# Autodesk Inventor assembly: Giant-Snes-Gamepad
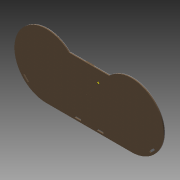
[picture p0: Inventor's stored thumbnail of the model, 180x180]
Saved by Autodesk Inventor 2014 SP1 (Build 180222100, 222)
## iProperties
Created: 2014-01-12
Part Number: Giant-Snes-Gamepad
Document SubType Name: Assembly
Designer: tuleu
Author: tuleu
## Documents named in this file (9)
- C:\Users\tuleu\Documents\giant-snes-gamepad\cad\Giant_Snes_Gamepad.iam
- C:\Users\tuleu\Documents\giant-snes-gamepad\cad\Base.ipt
- C:\Users\tuleu\Documents\giant-snes-gamepad\cad\Link.ipt
- C:\Users\tuleu\Documents\giant-snes-gamepad\cad\Square_Cell.iam
- C:\Users\tuleu\Documents\giant-snes-gamepad\cad\Trigger_Cell.iam
- C:\Users\tuleu\Documents\giant-snes-gamepad\cad\Foam_Left.ipt
- C:\Users\tuleu\Documents\giant-snes-gamepad\cad\Start_Cell.iam
- C:\Users\tuleu\Documents\giant-snes-gamepad\cad\Circle_Cell.iam
- C:\Users\tuleu\Documents\giant-snes-gamepad\cad\Foam_Right.ipt
## Components (19 placed, 8 different names)
1. Base:1 — Mate:1, Mate:2, Flush:1, Mate:3, Mate:5, Mate:6, Flush:3, Mate:15, Mate:16, Mate:17, Mate:18, Mate:20, Mate:21, Mate:22, Mate:24, Flush:22, Mate:29, Mate:31, Mate:32, Mate:33, Mate:35, Angle:1, Mate:37, Angle:2
2. Base:2 — Mate:1, Mate:2, Flush:1, Mate:3, Mate:4, Flush:2, Mate:10, Mate:11, Mate:12, Mate:13, Mate:27, Mate:28, Mate:30, Mate:34, Mate:38, Mate:39, Mate:40, Mate:41, Mate:42, Mate:43, Mate:46, Mate:47, Mate:48, Mate:49, Mate:50, Mate:51, Mate:53, Mate:54, Mate:55
3. Link:1 — Mate:4, Flush:2, Mate:12
4. Link:2 — Mate:5, Mate:10, Mate:14
5. Link:3 — Mate:6, Flush:3, Mate:11
6. Square_Cell:1 [sub-assembly] — Mate:17, Mate:19, Symmetry:2, Mate:20, Mate:23
7. Square_Cell:2 [sub-assembly] — Mate:15, Flush:21, Symmetry:1
8. Square_Cell:3 [sub-assembly] — Mate:16, Mate:19, Symmetry:2
9. Square_Cell:4 [sub-assembly] — Mate:18, Flush:21, Symmetry:1, Mate:21, Mate:22
10. Trigger_Cell:1 [sub-assembly] — Mate:24, Flush:22, Mate:29
11. Trigger_Cell:2 [sub-assembly] — Mate:27, Mate:28, Mate:30
12. Foam_Left:1 — Mate:31, Mate:32
13. Start_Cell:1 [sub-assembly] — Mate:33, Mate:36, Mate:37
14. Start_Cell:2 [sub-assembly] — Mate:34, Flush:23, Mate:39
15. Circle_Cell:1 [sub-assembly] — Mate:40, Mate:44, Mate:46, Mate:48
16. Circle_Cell:2 [sub-assembly] — Mate:41, Mate:45, Mate:47, Mate:50
17. Circle_Cell:3 [sub-assembly] — Mate:42, Mate:44, Mate:49
18. Circle_Cell:4 [sub-assembly] — Mate:43, Mate:45, Mate:51
19. Foam_Right:1 — Mate:53, Mate:54, Mate:55
## Relationships (59: Mate 49, Flush 6, Symmetry 2, Angle 2)
- Mate:1: Base:1 ↔ Base:2
- Mate:2: Base:1 ↔ Base:2
- Flush:1: Base:1 ↔ Base:2
- Mate:3: Base:1 ↔ Base:2
- Mate:4: Base:2 ↔ Link:1
- Mate:5: Base:1 ↔ Link:2
- Mate:6: Base:1 ↔ Link:3
- Flush:2: Base:2 ↔ Link:1
- Flush:3: Base:1 ↔ Link:3
- Mate:10: Base:2 ↔ Link:2
- Mate:11: Base:2 ↔ Link:3
- Mate:12: Base:2 ↔ Link:1
- Mate:13: Base:2
- Mate:14: Link:2
- Mate:15: Base:1 ↔ Square_Cell:2
- Mate:16: Base:1 ↔ Square_Cell:3
- Mate:17: Base:1 ↔ Square_Cell:1
- Mate:18: Base:1 ↔ Square_Cell:4
- Mate:19: Square_Cell:1 ↔ Square_Cell:3
- Flush:21: Square_Cell:2 ↔ Square_Cell:4
- Symmetry:1: Square_Cell:2 ↔ Square_Cell:4
- Symmetry:2: Square_Cell:1 ↔ Square_Cell:3
- Mate:20: Base:1 ↔ Square_Cell:1
- Mate:21: Base:1 ↔ Square_Cell:4
- Mate:22 (205 mm): Base:1 ↔ Square_Cell:4
- Mate:23 (-205 mm): Square_Cell:1
- Mate:24: Base:1 ↔ Trigger_Cell:1
- Mate:27: Base:2 ↔ Trigger_Cell:2
- Flush:22: Base:1 ↔ Trigger_Cell:1
- Mate:28: Base:2 ↔ Trigger_Cell:2
- Mate:29 (-400 mm): Base:1 ↔ Trigger_Cell:1
- Mate:30 (-400 mm): Base:2 ↔ Trigger_Cell:2
- Mate:31: Base:1 ↔ Foam_Left:1
- Mate:32: Base:1 ↔ Foam_Left:1
- Mate:33: Base:1 ↔ Start_Cell:1
- Mate:34: Base:2 ↔ Start_Cell:2
- Mate:35: Base:1
- Angle:1 (0 deg): Base:1
- Mate:36: Start_Cell:1
- Mate:37: Base:1 ↔ Start_Cell:1
- Mate:38: Base:2
- Angle:2 (0 deg): Base:1
- Flush:23: Start_Cell:2
- Mate:39: Base:2 ↔ Start_Cell:2
- Mate:40: Base:2 ↔ Circle_Cell:1
- Mate:41: Base:2 ↔ Circle_Cell:2
- Mate:42: Base:2 ↔ Circle_Cell:3
- Mate:43: Base:2 ↔ Circle_Cell:4
- Mate:44: Circle_Cell:1 ↔ Circle_Cell:3
- Mate:45: Circle_Cell:2 ↔ Circle_Cell:4
- Mate:46: Base:2 ↔ Circle_Cell:1
- Mate:47: Base:2 ↔ Circle_Cell:2
- Mate:48 (-280 mm): Base:2 ↔ Circle_Cell:1
- Mate:49 (-280 mm): Base:2 ↔ Circle_Cell:3
- Mate:50 (-280 mm): Base:2 ↔ Circle_Cell:2
- Mate:51 (-280 mm): Base:2 ↔ Circle_Cell:4
- Mate:53: Base:2 ↔ Foam_Right:1
- Mate:54: Base:2 ↔ Foam_Right:1
- Mate:55: Base:2 ↔ Foam_Right:1
